# Autodesk Inventor assembly: Assembly1_MIR
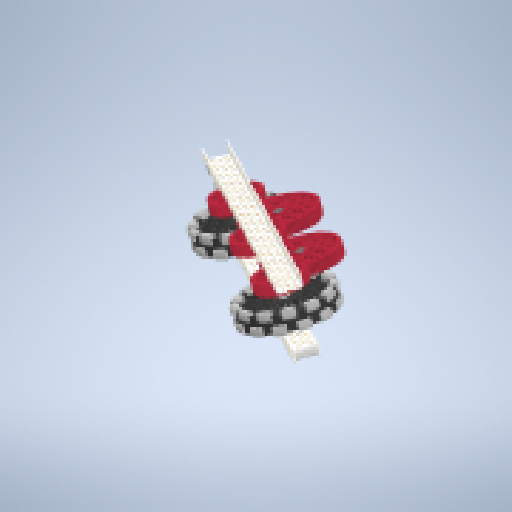
[picture p0: Inventor's stored thumbnail of the model, 512x512]
Saved by Autodesk Inventor 2024 (Build 280153000, 153)
## iProperties
Created: 2023-09-19
Part Number: Assembly1_MIR
Document SubType Name: Assembly
Designer: Robodox
Author: Robodox
## Documents named in this file (13)
- C:\Users\Robodox\Documents\GitHub\VEXCAD\Assembly1_MIR.iam
- C:\Users\Robodox\Documents\GitHub\VEX-CAD-Inventor\Structure\C Channel\Aluminum 1x2x1\Alu C 1x2x1x30_MIR.ipt
- C:\Users\Robodox\Documents\GitHub\VEXCAD\Part1_MIR.ipt
- C:\Users\Robodox\Documents\GitHub\VEXCAD\Part2_MIR1.ipt
- C:\Users\Robodox\Documents\GitHub\VEXCAD\Part3_MIR.ipt
- C:\Users\Robodox\Documents\GitHub\VEXCAD\Part5_MIR.ipt
- C:\Users\Robodox\Documents\GitHub\VEXCAD\Part4_MIR.ipt
- C:\Users\Robodox\Documents\GitHub\VEXCAD\part8_MIR.ipt
- C:\Users\Robodox\Documents\GitHub\VEX-CAD-Inventor\Motion\Wheels\Omni Wheel\4 Omni AS, Square_MIR.iam
- C:\Users\Robodox\Documents\GitHub\VEX-CAD-Inventor\Motion\Gears\HS Gear\HS 72T Gear, Square_MIR.iam
- C:\Users\Robodox\Documents\GitHub\VEX-CAD-Inventor\Motion\Gears\HS Gear\HS 48T Gear, Square_MIR.iam
- C:\Users\Robodox\Documents\GitHub\VEX-CAD-Inventor\Motion\Shaft LS\Bearing Flat_MIR.ipt
- C:\Users\Robodox\Documents\GitHub\VEX-CAD-Inventor\Motion\Shaft LS\LS Pillow Bearing Block_MIR.ipt
## Components (48 placed, 12 different names)
1. Alu C 1x2x1x30_MIR:1 — Flush:2, Flush:1, Mate:2, Mate:1, Mate:11, Mate:7, Mate:15, Mate:12, Mate:27, Mate:32, Mate:31, Mate:38, Mate:33, Mate:37, Mate:34, Mate:36, Mate:35, Mate:111, Mate:110, Mate:120, Mate:119, Mate:118, Mate:117, Mate:116, Mate:115, Mate:114, Mate:113, Mate:112
2. Alu C 1x2x1x30_MIR:2 — Flush:2, Flush:1, Mate:21, Mate:20, Mate:68, Mate:71, Mate:74
3. Part2_MIR1:3 — Mate:29, Mate:14, Mate:28, Mate:13
4. Part1_MIR:5 — Mate:29, Mate:14
5. Part1_MIR:6 — Mate:28, Mate:15, Mate:13, Mate:12
6. Part3_MIR:1 — Mate:32, Mate:31, Mate:125, Mate:121
7. Part3_MIR:2 — Mate:38, Mate:33, Mate:126
8. Part3_MIR:3 — Mate:37, Mate:34, Mate:123, Mate:122
9. Part3_MIR:4 — Mate:36, Mate:35, Mate:124
10. Part5_MIR:1 — Mate:52, Mate:47, Mate:96, Mate:94
11. Part5_MIR:2 — Mate:49, Mate:48, Mate:97, Mate:95
12. Part5_MIR:3 — Mate:52, Mate:47
13. Part5_MIR:4 — Mate:49, Mate:48
14. part8_MIR:1 — Mate:68, Mate:99, Mate:98
15. part8_MIR:2 — Mate:71, Mate:107, Mate:106
16. part8_MIR:3 — Mate:74, Mate:103, Mate:102
17. Part3_MIR:6 — Mate:90
18. Part3_MIR:7 — Mate:87, Mate:101, Mate:100
19. 4 Omni AS, Square_MIR:1 [sub-assembly] — Mate:87
20. 4 Omni AS, Square_MIR:2 [sub-assembly] — Mate:90
21. HS 72T Gear, Square_MIR:1 [sub-assembly] — Mate:96, Mate:94
22. HS 72T Gear, Square_MIR:2 [sub-assembly] — Mate:97, Mate:95
23. HS 48T Gear, Square_MIR:1 [sub-assembly] — Mate:99, Mate:98
24. HS 48T Gear, Square_MIR:2 [sub-assembly] — Mate:107, Mate:106, Mate:101, Mate:100
25. HS 48T Gear, Square_MIR:3 [sub-assembly] — Mate:103, Mate:102
26. Bearing Flat_MIR:1 — Mate:120, Mate:119, Mate:118
27. Bearing Flat_MIR:2 — Mate:117, Mate:116, Mate:115
28. Bearing Flat_MIR:3 — Mate:114, Mate:113, Mate:112
29. LS Pillow Bearing Block_MIR:1 — Mate:124, Mate:123, Mate:122
30. LS Pillow Bearing Block_MIR:2 — Mate:126, Mate:125, Mate:121
31. Part4_MIR:1 — Mate:27, Mate:25
32. Part3_MIR:5 — Mate:21, Mate:20, Mate:25
33. Part1_MIR:1 — Mate:5, Mate:4
34. Part2_MIR1:1 — Mate:5, Mate:4, Mate:6, Mate:3
35. Part1_MIR:2 — Mate:6, Mate:3, Mate:2, Mate:1
36. Part1_MIR:8
37. Part2_MIR1:5
38. Part1_MIR:9
39. Part1_MIR:3 — Mate:10, Mate:9
40. Part2_MIR1:2 — Mate:30, Mate:10, Mate:9, Mate:8
41. Part1_MIR:4 — Mate:11, Mate:7, Mate:30, Mate:8
42. Part1_MIR:10
43. Part2_MIR1:6
44. Part1_MIR:11
45. Part1_MIR:7 — Mate:111, Mate:110, Mate:109, Mate:108
46. Part2_MIR1:4 — Mate:109, Mate:108
47. Part1_MIR:12
48. Part2_MIR1:7
## Component patterns: (2 elements, first: Part1_MIR:1 + Part2_MIR1:1 + Part1_MIR:2), (2 elements, first: Part1_MIR:3 + Part2_MIR1:2 + Part1_MIR:4), (2 elements, first: Part1_MIR:7 + Part2_MIR1:4)
## Relationships (72: Mate 70, Flush 2)
- Flush:2: Alu C 1x2x1x30_MIR:1 ↔ Alu C 1x2x1x30_MIR:2
- Flush:1: Alu C 1x2x1x30_MIR:1 ↔ Alu C 1x2x1x30_MIR:2
- Mate:5: Part1_MIR:1 ↔ Part2_MIR1:1
- Mate:4: Part1_MIR:1 ↔ Part2_MIR1:1
- Mate:6: Part2_MIR1:1 ↔ Part1_MIR:2
- Mate:3: Part2_MIR1:1 ↔ Part1_MIR:2
- Mate:2: Alu C 1x2x1x30_MIR:1 ↔ Part1_MIR:2
- Mate:1: Alu C 1x2x1x30_MIR:1 ↔ Part1_MIR:2
- Mate:11: Alu C 1x2x1x30_MIR:1 ↔ Part1_MIR:4
- Mate:7: Alu C 1x2x1x30_MIR:1 ↔ Part1_MIR:4
- Mate:30: Part2_MIR1:2 ↔ Part1_MIR:4
- Mate:10: Part1_MIR:3 ↔ Part2_MIR1:2
- Mate:9: Part1_MIR:3 ↔ Part2_MIR1:2
- Mate:8: Part2_MIR1:2 ↔ Part1_MIR:4
- Mate:29: Part2_MIR1:3 ↔ Part1_MIR:5
- Mate:14: Part2_MIR1:3 ↔ Part1_MIR:5
- Mate:28: Part2_MIR1:3 ↔ Part1_MIR:6
- Mate:15: Alu C 1x2x1x30_MIR:1 ↔ Part1_MIR:6
- Mate:13: Part2_MIR1:3 ↔ Part1_MIR:6
- Mate:12: Alu C 1x2x1x30_MIR:1 ↔ Part1_MIR:6
- Mate:21: Alu C 1x2x1x30_MIR:2 ↔ Part3_MIR:5
- Mate:20: Alu C 1x2x1x30_MIR:2 ↔ Part3_MIR:5
- Mate:27: Alu C 1x2x1x30_MIR:1 ↔ Part4_MIR:1
- Mate:25: Part4_MIR:1 ↔ Part3_MIR:5
- Mate:32: Alu C 1x2x1x30_MIR:1 ↔ Part3_MIR:1
- Mate:31: Alu C 1x2x1x30_MIR:1 ↔ Part3_MIR:1
- Mate:38: Alu C 1x2x1x30_MIR:1 ↔ Part3_MIR:2
- Mate:33: Alu C 1x2x1x30_MIR:1 ↔ Part3_MIR:2
- Mate:37: Alu C 1x2x1x30_MIR:1 ↔ Part3_MIR:3
- Mate:34: Alu C 1x2x1x30_MIR:1 ↔ Part3_MIR:3
- Mate:36: Alu C 1x2x1x30_MIR:1 ↔ Part3_MIR:4
- Mate:35: Alu C 1x2x1x30_MIR:1 ↔ Part3_MIR:4
- Mate:52: Part5_MIR:1 ↔ Part5_MIR:3
- Mate:47: Part5_MIR:1 ↔ Part5_MIR:3
- Mate:49: Part5_MIR:2 ↔ Part5_MIR:4
- Mate:48: Part5_MIR:2 ↔ Part5_MIR:4
- Mate:68: Alu C 1x2x1x30_MIR:2 ↔ part8_MIR:1
- Mate:71: Alu C 1x2x1x30_MIR:2 ↔ part8_MIR:2
- Mate:74: Alu C 1x2x1x30_MIR:2 ↔ part8_MIR:3
- Mate:87: Part3_MIR:7 ↔ 4 Omni AS, Square_MIR:1
- Mate:90: Part3_MIR:6 ↔ 4 Omni AS, Square_MIR:2
- Mate:96: Part5_MIR:1 ↔ HS 72T Gear, Square_MIR:1
- Mate:94: Part5_MIR:1 ↔ HS 72T Gear, Square_MIR:1
- Mate:97: Part5_MIR:2 ↔ HS 72T Gear, Square_MIR:2
- Mate:95: Part5_MIR:2 ↔ HS 72T Gear, Square_MIR:2
- Mate:99: part8_MIR:1 ↔ HS 48T Gear, Square_MIR:1
- Mate:98: part8_MIR:1 ↔ HS 48T Gear, Square_MIR:1
- Mate:107: part8_MIR:2 ↔ HS 48T Gear, Square_MIR:2
- Mate:106: part8_MIR:2 ↔ HS 48T Gear, Square_MIR:2
- Mate:101: Part3_MIR:7 ↔ HS 48T Gear, Square_MIR:2
- Mate:100: Part3_MIR:7 ↔ HS 48T Gear, Square_MIR:2
- Mate:103: part8_MIR:3 ↔ HS 48T Gear, Square_MIR:3
- Mate:102: part8_MIR:3 ↔ HS 48T Gear, Square_MIR:3
- Mate:111: Alu C 1x2x1x30_MIR:1 ↔ Part1_MIR:7
- Mate:110: Alu C 1x2x1x30_MIR:1 ↔ Part1_MIR:7
- Mate:109: Part1_MIR:7 ↔ Part2_MIR1:4
- Mate:108: Part1_MIR:7 ↔ Part2_MIR1:4
- Mate:120: Alu C 1x2x1x30_MIR:1 ↔ Bearing Flat_MIR:1
- Mate:119: Alu C 1x2x1x30_MIR:1 ↔ Bearing Flat_MIR:1
- Mate:118: Alu C 1x2x1x30_MIR:1 ↔ Bearing Flat_MIR:1
- Mate:117: Alu C 1x2x1x30_MIR:1 ↔ Bearing Flat_MIR:2
- Mate:116: Alu C 1x2x1x30_MIR:1 ↔ Bearing Flat_MIR:2
- Mate:115: Alu C 1x2x1x30_MIR:1 ↔ Bearing Flat_MIR:2
- Mate:114: Alu C 1x2x1x30_MIR:1 ↔ Bearing Flat_MIR:3
- Mate:113: Alu C 1x2x1x30_MIR:1 ↔ Bearing Flat_MIR:3
- Mate:112: Alu C 1x2x1x30_MIR:1 ↔ Bearing Flat_MIR:3
- Mate:124: Part3_MIR:4 ↔ LS Pillow Bearing Block_MIR:1
- Mate:123: Part3_MIR:3 ↔ LS Pillow Bearing Block_MIR:1
- Mate:122: Part3_MIR:3 ↔ LS Pillow Bearing Block_MIR:1
- Mate:126: Part3_MIR:2 ↔ LS Pillow Bearing Block_MIR:2
- Mate:125: Part3_MIR:1 ↔ LS Pillow Bearing Block_MIR:2
- Mate:121: Part3_MIR:1 ↔ LS Pillow Bearing Block_MIR:2
